# Autodesk Inventor assembly: FinalAssemblyMerge
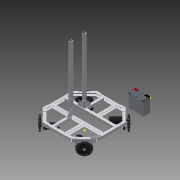
[picture p0: Inventor's stored thumbnail of the model, 180x180]
Saved by Autodesk Inventor 2015 (Build 190159000, 159)
## iProperties
Created: 2015-01-27
Part Number: FinalAssemblyMerge
Document SubType Name: Assembly
Designer: pltwe4
Author: pltwe4
## Documents named in this file (14)
- F:\CAD Models\Robotics BenT\Final Assembly.iam
- F:\CAD Models\Robotics BenT\NCornerChannel.ipt
- F:\CAD Models\Robotics BenT\NSideChannel.ipt
- F:\CAD Models\Robotics BenT\6-omni-wheel.iam
- F:\CAD Models\Robotics BenT\CornerBracket.ipt
- F:\CAD Models\Robotics BenT\NSupportChannel.ipt
- F:\CAD Models\Robotics BenT\AllowedEnvelope.ipt
- F:\CAD Models\Robotics BenT\NSupportChannel2.ipt
- F:\CAD Models\Robotics BenT\CimpleLeft.iam
- F:\CAD Models\Robotics BenT\CimpleRight.iam
- F:\CAD Models\Robotics BenT\Battery.iam
- F:\CAD Models\Robotics BenT\VerticalCorner.ipt
- F:\CAD Models\Robotics BenT\CornerBracketSheetMetal.ipt
- F:\CAD Models\Robotics BenT\NTowerChannel2.ipt
## Components (45 placed, 13 different names)
1. AllowedEnvelope:1 — Flush:52, Mate:114
2. Battery:1 [sub-assembly]
3. CornerBracketSheetMetal:1 — Mate:119, Flush:80, Flush:81
4. VerticalCorner:1 — Flush:82, Flush:83, Flush:84, Mate:121, Mate:122, Mate:123
5. VerticalCorner:2 — Mate:120, Flush:82, Flush:85, Flush:86, Mate:124, Mate:125, Mate:126
6. NTowerChannel2:1 — Mate:121, Mate:122, Mate:123
7. NTowerChannel2:2 — Mate:124, Mate:125, Mate:126
8. NSupportChannel:1 — Mate:65, Flush:51, Mate:69, Flush:57, Mate:80, Mate:120, Flush:85
9. NSupportChannel:2 — Mate:36, Mate:37, Flush:47, Flush:53, Mate:67, Mate:68, Flush:83
10. NSupportChannel2:1 — Flush:53, Flush:54, Flush:56, Mate:67, Mate:73, Flush:84
11. NSupportChannel2:6 — Flush:57, Mate:76, Mate:77, Mate:80, Flush:86
12. NSupportChannel2:4 — Flush:56, Mate:69, Mate:75
13. NSupportChannel2:2 — Flush:54, Mate:68, Mate:72, Mate:74
14. NSideChannel:2 — Flush:45, Mate:46, Mate:49, Mate:52, Flush:49, Mate:59, Mate:72, Mate:117
15. NSideChannel:3 — Mate:37, Flush:47, Mate:45, Mate:51, Flush:50, Mate:74, Mate:75, Mate:82, Mate:85, Mate:119, Flush:80
16. NSideChannel:4 — Mate:41, Mate:42, Mate:52, Flush:49, Mate:64, Mate:76, Mate:81
17. NSideChannel:1 — Flush:3, Mate:4, Mate:5, Flush:7, Mate:6, Mate:7, Flush:10, Flush:21, Mate:15, Mate:36, Flush:50, Mate:57, Mate:58, Mate:63, Mate:65, Flush:51, Mate:73, Mate:77
18. NCornerChannel:1 — Flush:3, Flush:6, Mate:16, Flush:48, Mate:39, Mate:40, Angle:10, Flush:63, Flush:67
19. NCornerChannel:2 — Flush:21, Flush:22, Mate:38, Mate:47, Mate:56, Angle:9, Flush:62, Flush:68
20. NCornerChannel:3 — Flush:45, Flush:46, Mate:39, Mate:44, Mate:48, Flush:64, Flush:65, Mate:118, Flush:81
21. NCornerChannel:4 — Mate:38, Mate:43, Mate:50, Flush:61, Flush:66
22. 6-omni-wheel:1 [sub-assembly] — Mate:89, Mate:92
23. 6-omni-wheel:2 [sub-assembly] — Mate:88, Mate:93
24. 6-omni-wheel:3 [sub-assembly] — Mate:87, Mate:90
25. 6-omni-wheel:4 [sub-assembly] — Mate:86, Mate:91
26. CornerBracket:1 — Mate:5, Flush:4, Flush:5
27. CornerBracket:2 — Mate:4, Flush:4, Flush:5, Flush:6, Flush:7, Angle:1
28. CornerBracket:3 — Mate:7, Flush:8, Flush:9
29. CornerBracket:4 — Mate:6, Flush:8, Flush:9, Flush:10, Flush:22, Angle:8
30. CornerBracket:5
31. CornerBracket:6 — Angle:5
32. CornerBracket:7
33. CornerBracket:8 — Flush:46, Angle:6
34. CornerBracket:9
35. CornerBracket:10 — Angle:4
36. CornerBracket:11
37. CornerBracket:12 — Angle:7
38. CornerBracket:13
39. CornerBracket:14 — Angle:3
40. CornerBracket:15
41. CornerBracket:16 — Flush:48, Angle:2
42. CimpleLeft:1 [sub-assembly] — Flush:58, Mate:85, Flush:62, Flush:68, Mate:88, Mate:93
43. CimpleRight:1 [sub-assembly] — Flush:58, Flush:59, Flush:60, Flush:64, Flush:65, Mate:87, Mate:90, Mate:94
44. CimpleLeft:2 [sub-assembly] — Flush:59, Flush:61, Flush:66, Mate:86, Mate:91
45. CimpleRight:2 [sub-assembly] — Flush:60, Flush:63, Flush:67, Mate:89, Mate:92
## Relationships (154: Mate 78, Flush 66, Angle 10)
- Flush:3: NSideChannel:1 ↔ NCornerChannel:1
- Mate:4: NSideChannel:1 ↔ CornerBracket:2
- Mate:5: NSideChannel:1 ↔ CornerBracket:1
- Flush:4: CornerBracket:1 ↔ CornerBracket:2
- Flush:5: CornerBracket:1 ↔ CornerBracket:2
- Flush:6: NCornerChannel:1 ↔ CornerBracket:2
- Flush:7: NSideChannel:1 ↔ CornerBracket:2
- Mate:6: NSideChannel:1 ↔ CornerBracket:4
- Mate:7: NSideChannel:1 ↔ CornerBracket:3
- Flush:8: CornerBracket:3 ↔ CornerBracket:4
- Flush:9: CornerBracket:3 ↔ CornerBracket:4
- Flush:10: NSideChannel:1 ↔ CornerBracket:4
- [Flush]: NSideChannel:2 ↔ NCornerChannel:2
- [Mate]: NSideChannel:2 ↔ CornerBracket:6
- [Mate]: NSideChannel:2 ↔ CornerBracket:5
- [Flush]: CornerBracket:5 ↔ CornerBracket:6
- [Flush]: CornerBracket:5 ↔ CornerBracket:6
- [Flush]: NCornerChannel:2 ↔ CornerBracket:6
- [Flush]: NSideChannel:2 ↔ CornerBracket:6
- [Mate]: NSideChannel:2 ↔ CornerBracket:8
- [Mate]: NSideChannel:2 ↔ CornerBracket:7
- [Flush]: CornerBracket:7 ↔ CornerBracket:8
- [Flush]: CornerBracket:7 ↔ CornerBracket:8
- [Flush]: NSideChannel:2 ↔ CornerBracket:8
- Flush:21: NSideChannel:1 ↔ NCornerChannel:2
- Flush:22: NCornerChannel:2 ↔ CornerBracket:4
- Mate:15: NSideChannel:1
- Mate:16: NCornerChannel:1
- Angle:1 (90 deg): CornerBracket:2
- [Flush]: NSideChannel:3 ↔ NCornerChannel:3
- [Mate]: NSideChannel:3 ↔ CornerBracket:10
- [Mate]: NSideChannel:3 ↔ CornerBracket:9
- [Flush]: CornerBracket:9 ↔ CornerBracket:10
- [Flush]: CornerBracket:9 ↔ CornerBracket:10
- [Flush]: NCornerChannel:3 ↔ CornerBracket:10
- [Flush]: NSideChannel:3 ↔ CornerBracket:10
- [Mate]: NSideChannel:3 ↔ CornerBracket:12
- [Mate]: NSideChannel:3 ↔ CornerBracket:11
- [Flush]: CornerBracket:11 ↔ CornerBracket:12
- [Flush]: CornerBracket:11 ↔ CornerBracket:12
- [Flush]: NSideChannel:3 ↔ CornerBracket:12
- [Flush]: NSideChannel:4 ↔ NCornerChannel:4
- [Mate]: NSideChannel:4 ↔ CornerBracket:14
- [Mate]: NSideChannel:4 ↔ CornerBracket:13
- [Flush]: CornerBracket:13 ↔ CornerBracket:14
- [Flush]: CornerBracket:13 ↔ CornerBracket:14
- [Flush]: NCornerChannel:4 ↔ CornerBracket:14
- [Flush]: NSideChannel:4 ↔ CornerBracket:14
- [Mate]: NSideChannel:4 ↔ CornerBracket:16
- [Mate]: NSideChannel:4 ↔ CornerBracket:15
- [Flush]: CornerBracket:15 ↔ CornerBracket:16
- [Flush]: CornerBracket:15 ↔ CornerBracket:16
- [Flush]: NSideChannel:4 ↔ CornerBracket:16
- [Flush]: NSideChannel:3 ↔ NCornerChannel:4
- [Flush]: NCornerChannel:4 ↔ CornerBracket:12
- Flush:45: NSideChannel:2 ↔ NCornerChannel:3
- Flush:46: NCornerChannel:3 ↔ CornerBracket:8
- Mate:36: NSupportChannel:2 ↔ NSideChannel:1
- Mate:37: NSupportChannel:2 ↔ NSideChannel:3
- Flush:47: NSupportChannel:2 ↔ NSideChannel:3
- Flush:48: NCornerChannel:1 ↔ CornerBracket:16
- Mate:38: NCornerChannel:2 ↔ NCornerChannel:4
- Mate:39: NCornerChannel:1 ↔ NCornerChannel:3
- Mate:40: NCornerChannel:1
- Mate:41: NSideChannel:4
- Angle:2 (90 deg): CornerBracket:16
- Mate:42: NSideChannel:4
- Mate:43: NCornerChannel:4
- Angle:3 (90 deg): CornerBracket:14
- Mate:44: NCornerChannel:3
- Mate:45: NSideChannel:3
- Angle:4 (90 deg): CornerBracket:10
- Mate:46: NSideChannel:2
- Mate:47: NCornerChannel:2
- Angle:5 (90 deg): CornerBracket:6
- Mate:48: NCornerChannel:3
- Mate:49: NSideChannel:2
- Angle:6 (90 deg): CornerBracket:8
- Mate:50: NCornerChannel:4
- Mate:51: NSideChannel:3
- Angle:7 (90 deg): CornerBracket:12
- Mate:52 (584.2 mm): NSideChannel:2 ↔ NSideChannel:4
- Flush:49: NSideChannel:2 ↔ NSideChannel:4
- Flush:50: NSideChannel:3 ↔ NSideChannel:1
- Mate:56: NCornerChannel:2
- Mate:57: NSideChannel:1
- Angle:8 (90 deg): CornerBracket:4
- Mate:58: NSideChannel:1
- Mate:59: NSideChannel:2
- Angle:9 (0 deg): NCornerChannel:2
- Mate:60
- Mate:61
- Mate:62
- Mate:63: NSideChannel:1
- Mate:64: NSideChannel:4
- Angle:10 (0 deg): NCornerChannel:1
- Mate:65: NSupportChannel:1 ↔ NSideChannel:1
- Flush:51: NSupportChannel:1 ↔ NSideChannel:1
- Flush:52: AllowedEnvelope:1
- Flush:53: NSupportChannel:2 ↔ NSupportChannel2:1
- Flush:54: NSupportChannel2:1 ↔ NSupportChannel2:2
- Flush:56: NSupportChannel2:1 ↔ NSupportChannel2:4
- Mate:67: NSupportChannel:2 ↔ NSupportChannel2:1
- Mate:68: NSupportChannel:2 ↔ NSupportChannel2:2
- Mate:69: NSupportChannel:1 ↔ NSupportChannel2:4
- Mate:72: NSupportChannel2:2 ↔ NSideChannel:2
- Mate:73 (203.2 mm): NSupportChannel2:1 ↔ NSideChannel:1
- Mate:74 (203.2 mm): NSupportChannel2:2 ↔ NSideChannel:3
- Mate:75 (203.2 mm): NSupportChannel2:4 ↔ NSideChannel:3
- Flush:57: NSupportChannel:1 ↔ NSupportChannel2:6
- Mate:76: NSupportChannel2:6 ↔ NSideChannel:4
- Mate:77 (203.2 mm): NSupportChannel2:6 ↔ NSideChannel:1
- Mate:80: NSupportChannel:1 ↔ NSupportChannel2:6
- Mate:81: NSideChannel:4
- Mate:82: NSideChannel:3
- Flush:58: CimpleLeft:1 ↔ CimpleRight:1
- Flush:59: CimpleRight:1 ↔ CimpleLeft:2
- Flush:60: CimpleRight:1 ↔ CimpleRight:2
- Mate:85: NSideChannel:3 ↔ CimpleLeft:1
- Flush:61: NCornerChannel:4 ↔ CimpleLeft:2
- Flush:62: NCornerChannel:2 ↔ CimpleLeft:1
- Flush:63: NCornerChannel:1 ↔ CimpleRight:2
- Flush:64: NCornerChannel:3 ↔ CimpleRight:1
- Flush:65: NCornerChannel:3 ↔ CimpleRight:1
- Flush:66: NCornerChannel:4 ↔ CimpleLeft:2
- Flush:67: NCornerChannel:1 ↔ CimpleRight:2
- Flush:68: NCornerChannel:2 ↔ CimpleLeft:1
- Mate:86: 6-omni-wheel:4 ↔ CimpleLeft:2
- Mate:87: 6-omni-wheel:3 ↔ CimpleRight:1
- Mate:88: 6-omni-wheel:2 ↔ CimpleLeft:1
- Mate:89: 6-omni-wheel:1 ↔ CimpleRight:2
- Mate:90 (12.7 mm): 6-omni-wheel:3 ↔ CimpleRight:1
- Mate:91 (12.7 mm): 6-omni-wheel:4 ↔ CimpleLeft:2
- Mate:92 (12.7 mm): 6-omni-wheel:1 ↔ CimpleRight:2
- Mate:93 (12.7 mm): 6-omni-wheel:2 ↔ CimpleLeft:1
- Mate:94 (76.2 mm): CimpleRight:1
- Mate:114: AllowedEnvelope:1
- Mate:117: NSideChannel:2
- Mate:118: NCornerChannel:3
- Mate:119: CornerBracketSheetMetal:1 ↔ NSideChannel:3
- Flush:80: CornerBracketSheetMetal:1 ↔ NSideChannel:3
- Flush:81: CornerBracketSheetMetal:1 ↔ NCornerChannel:3
- Mate:120: VerticalCorner:2 ↔ NSupportChannel:1
- Flush:82: VerticalCorner:1 ↔ VerticalCorner:2
- Flush:83: VerticalCorner:1 ↔ NSupportChannel:2
- Flush:84: VerticalCorner:1 ↔ NSupportChannel2:1
- Flush:85: VerticalCorner:2 ↔ NSupportChannel:1
- Flush:86: VerticalCorner:2 ↔ NSupportChannel2:6
- Mate:121: VerticalCorner:1 ↔ NTowerChannel2:1
- Mate:122: VerticalCorner:1 ↔ NTowerChannel2:1
- Mate:123: VerticalCorner:1 ↔ NTowerChannel2:1
- Mate:124: VerticalCorner:2 ↔ NTowerChannel2:2
- Mate:125: VerticalCorner:2 ↔ NTowerChannel2:2
- Mate:126: VerticalCorner:2 ↔ NTowerChannel2:2
## Named parameters: Tolerance = 0 mm, Hub2Wheel = 12.7 mm, d17_d11 = 0 mm, d18_d12 = 0 mm, d19_d13 = 0 mm, d20_d14 = 0 mm, d21_d15 = 0 mm, d22_d16 = 0 mm, d27_d5 = 0 mm, d28_d6 = 0 mm, d29_d7 = 0 mm, d30_d8 = 0 mm, d31_d9 = 0 mm, d32_d10 = 0 mm, d43_d35 = 0 mm, d44_d36 = 0 mm, d48_d11 = 0 mm, d49_d12 = 0 mm, d50_d13 = 0 mm, d51_d14 = 0 mm, d52_d15 = 0 mm, d53_d16 = 0 mm, d54_d17_d11 = 0 mm, d55_d18_d12 = 0 mm, d56_d19_d13 = 0 mm, d57_d20_d14 = 0 mm, d58_d21_d15 = 0 mm, d59_d22_d16 = 0 mm, d64_d27_d5 = 0 mm, d65_d28_d6 = 0 mm, d66_d29_d7 = 0 mm, d67_d30_d8 = 0 mm, d68_d31_d9 = 0 mm, d69_d32_d10 = 0 mm, d76_d5 = 0 mm, d77_d6 = 0 mm, d78_d7 = 0 mm, d79_d8 = 0 mm, d80_d9 = 0 mm, d81_d10 = 0 mm, SupportLength = 584.2 mm, Support2Length = 203.2 mm
